# Autodesk Inventor assembly: pneumaticTestBoard
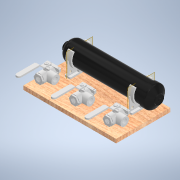
[picture p0: Inventor's stored thumbnail of the model, 180x180]
Saved by Autodesk Inventor 2020.2 (Build 242310000, 310)
## iProperties
Created: 2020-01-23
Part Number: pneumaticTestBoard
Document SubType Name: Assembly
Designer: robst
Author: robst
## Documents named in this file (5)
- C:\git\CAD-Development\robSteele\2020PneumaticTestBoard\pneumaticTestBoard.iam
- C:\git\CAD-Development\robSteele\2020PneumaticTestBoard\fc18-082_AirVolTank.ipt
- C:\git\CAD-Development\robSteele\2020PneumaticTestBoard\am-2008-bracket.ipt
- C:\git\CAD-Development\robSteele\2020PneumaticTestBoard\4373K510_DIVERTING 3-PORT BRONZE BALL VALVE.ipt
- C:\git\CAD-Development\robSteele\2020PneumaticTestBoard\plywoodBasePlate.ipt
## Components (7 placed, 4 different names)
1. plywoodBasePlate:1 — Insert:1, Insert:2
2. fc18-082_AirVolTank:1 — Insert:3
3. am-2008-bracket:1 — Insert:1
4. am-2008-bracket:2 — Insert:2, Insert:3
5. 4373K510_DIVERTING 3-PORT BRONZE BALL VALVE:1
6. 4373K510_DIVERTING 3-PORT BRONZE BALL VALVE:2
7. 4373K510_DIVERTING 3-PORT BRONZE BALL VALVE:3
## Relationships (3: Insert 3)
- Insert:1: plywoodBasePlate:1 ↔ am-2008-bracket:1
- Insert:2: plywoodBasePlate:1 ↔ am-2008-bracket:2
- Insert:3 (50.8 mm): fc18-082_AirVolTank:1 ↔ am-2008-bracket:2
